# Autodesk Inventor assembly: ForeArm
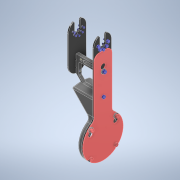
[picture p0: Inventor's stored thumbnail of the model, 180x180]
Saved by Autodesk Inventor 2022 (Build 260153000, 153)
## iProperties
Created: 2023-06-02
Part Number: ForeArm
Document SubType Name: Assembly
Designer: Masato Kubotera
Mass: 139.632 g
Surface Area: 907.343 cm^2
Volume: 92.9837 cm^3
Density: 1.50168 g/cm^3
Author: Masato Kubotera
## Documents named in this file (3)
- C:\Users\MasatoKubotera\Documents\Inventor\SUSTAINA-OP\UpperBody\Arm\ForeArm.iam
- C:\Users\MasatoKubotera\Documents\Inventor\SUSTAINA-OP\UpperBody\Arm\ForeArm_without_hand.iam
- C:\Users\MasatoKubotera\Documents\Inventor\SUSTAINA-OP\UpperBody\Arm\ForeArm_hand.iam
## Components (2 placed, 2 different names)
1. ForeArm_without_hand:1 [sub-assembly] — Insert:1, Insert:2, Insert:3, Insert:4, フラッシュ:1, フラッシュ:2, フラッシュ:3
2. ForeArm_hand:1 [sub-assembly] — Insert:1, Insert:2, Insert:3, Insert:4
## Relationships (7: Insert 4, Flush 3)
- Insert:1: ForeArm_without_hand:1 ↔ ForeArm_hand:1
- Insert:2: ForeArm_without_hand:1 ↔ ForeArm_hand:1
- Insert:3: ForeArm_without_hand:1 ↔ ForeArm_hand:1
- Insert:4: ForeArm_without_hand:1 ↔ ForeArm_hand:1
- フラッシュ:1 [Flush]: ForeArm_without_hand:1
- フラッシュ:2 [Flush]: ForeArm_without_hand:1
- フラッシュ:3 [Flush]: ForeArm_without_hand:1
